# Autodesk Inventor assembly: 0005-00-02 X axis
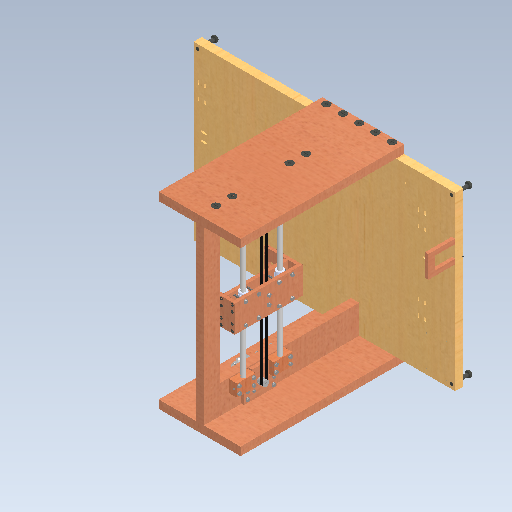
[picture p0: Inventor's stored thumbnail of the model, 512x512]
Saved by Autodesk Inventor 2020 (Build 240168000, 168)
## iProperties
Created: 2020-12-18
Part Number: 0005-00-02 X axis
Document SubType Name: Assembly
Designer: Iulian Bors
Mass: 798.511 g
Surface Area: 2520.75 cm^2
Volume: 569.854 cm^3
Density: 1.40126 g/cm^3
Author: Iulian Bors
Subject: 10-02
## Documents named in this file (22)
- Z:\I.A.B\Proiecte\0005 I.A.B 3d 2.0 Imprimanta aracet\10 Mecanic\0005-10-02 X axis.iam
- Z:\I.A.B\Proiecte\0005 I.A.B 3d 2.0 Imprimanta aracet\10 Mecanic\0005-10-011.ipt
- Z:\I.A.B\Proiecte\0005 I.A.B 3d 2.0 Imprimanta aracet\10 Mecanic\0005-10-012.ipt
- Z:\I.A.B\Proiecte\0005 I.A.B 3d 2.0 Imprimanta aracet\10 Mecanic\0005-10-1009 LM10uu.ipt
- Z:\I.A.B\Proiecte\0005 I.A.B 3d 2.0 Imprimanta aracet\10 Mecanic\Surub M4 saiba piulita.iam
- Z:\I.A.B\Proiecte\0005 I.A.B 3d 2.0 Imprimanta aracet\10 Mecanic\0005-10-1007 Bara rectificata.ipt
- Z:\I.A.B\Proiecte\0005 I.A.B 3d 2.0 Imprimanta aracet\10 Mecanic\0005-10-015 suport tija.ipt
- Z:\I.A.B\Proiecte\0005 I.A.B 3d 2.0 Imprimanta aracet\10 Mecanic\0005-10-1001 NEMA17 - Motor de passo.ipt
- Z:\I.A.B\Proiecte\0005 I.A.B 3d 2.0 Imprimanta aracet\10 Mecanic\0005-10-1010 GT2 Timing Pulley 20 Tooth.ipt
- Z:\I.A.B\Proiecte\0005 I.A.B 3d 2.0 Imprimanta aracet\10 Mecanic\0005-10-1011 16T W6 B3 Without T_Shrinkwrap_1.ipt
- Z:\I.A.B\Proiecte\0005 I.A.B 3d 2.0 Imprimanta aracet\10 Mecanic\0005-10-018 intinzator x.ipt
- Z:\I.A.B\Proiecte\0005 I.A.B 3d 2.0 Imprimanta aracet\10 Mecanic\0005-10-1015 curea x.ipt
- Z:\I.A.B\Proiecte\0005 I.A.B 3d 2.0 Imprimanta aracet\10 Mecanic\0005-10-023 Suport motor x.ipt
- Z:\I.A.B\Proiecte\0005 I.A.B 3d 2.0 Imprimanta aracet\10 Mecanic\Surub M4 saiba piulita 50mm.iam
- Z:\I.A.B\Proiecte\0005 I.A.B 3d 2.0 Imprimanta aracet\10 Mecanic\Surub M4 saiba piulita 60mm.iam
- Z:\I.A.B\Proiecte\0005 I.A.B 3d 2.0 Imprimanta aracet\10 Mecanic\0005-10-1032.ipt
- Z:\I.A.B\Proiecte\0005 I.A.B 3d 2.0 Imprimanta aracet\10 Mecanic\0005-10-1020 ISO 7089 - 3 - 140 HV(1).ipt
- Z:\I.A.B\Proiecte\0005 I.A.B 3d 2.0 Imprimanta aracet\10 Mecanic\0005-10-1033 DIN 914 - M5 x 10.ipt
- Z:\I.A.B\Proiecte\0005 I.A.B 3d 2.0 Imprimanta aracet\10 Mecanic\0005-10-027 suport nema Z.ipt
- Z:\I.A.B\Proiecte\0005 I.A.B 3d 2.0 Imprimanta aracet\10 Mecanic\0005-10-01 Cadru_Shrinkwrap_1.ipt
- Z:\I.A.B\Proiecte\0005 I.A.B 3d 2.0 Imprimanta aracet\10 Mecanic\0005-10-1045ISO 7050 - ST 3.5 x 22 - C - Z.ipt
- Z:\I.A.B\Proiecte\0005 I.A.B 3d 2.0 Imprimanta aracet\10 Mecanic\0005-10-1048 DIN 933 - M5  x 25.ipt
## Components (82 placed, 21 different names)
1. 0005-10-011.ipt:1 — Flush:69, Flush:70, Mate:151, Insert:33, Insert:34
2. 0005-10-027 suport nema Z.ipt:2 — Mate:142, Flush:71, Flush:72, Insert:35, Insert:36
3. 0005-10-012.ipt:3 — Flush:22, Flush:25, Flush:26, Mate:40, Mate:56, Mate:57, Mate:71, Mate:72, Flush:44, Mate:142, Mate:151
4. 0005-10-1009 LM10uu.ipt:4 — Flush:22, Mate:49, Mate:56, Mate:57
5. 0005-10-012.ipt:5 — Flush:25, Flush:34, Flush:26, Mate:40, Insert:18, Insert:19, Flush:69, Flush:70, Flush:71, Flush:72, Insert:21, Insert:22, Insert:24, Insert:25, Insert:27, Insert:28, Insert:30, Insert:40
6. 0005-10-1009 LM10uu.ipt:6 — Mate:49, Flush:34, Flush:45, Mate:172
7. 0005-10-1009 LM10uu.ipt:7 — Mate:71, Mate:72, Flush:44, Mate:73
8. 0005-10-1009 LM10uu.ipt:8 — Flush:45, Mate:73, Mate:164
9. Surub M4 saiba piulita.iam:9 [sub-assembly] — Insert:18
10. Surub M4 saiba piulita.iam:10 [sub-assembly] — Insert:19
11. Surub M4 saiba piulita.iam:11 [sub-assembly] — Insert:21
12. Surub M4 saiba piulita.iam:12 [sub-assembly] — Insert:22
13. Surub M4 saiba piulita.iam:13 [sub-assembly] — Insert:24
14. Surub M4 saiba piulita.iam:14 [sub-assembly] — Insert:27
15. Surub M4 saiba piulita.iam:15 [sub-assembly] — Insert:25
16. Surub M4 saiba piulita.iam:16 [sub-assembly] — Insert:28
17. Surub M4 saiba piulita.iam:17 [sub-assembly] — Insert:30
18. 0005-10-1007 Bara rectificata.ipt:18 — Mate:172, Mate:173, Flush:75, Mate:176, Flush:77
19. 0005-10-015 suport tija.ipt:19 — Mate:165, Mate:166, Mate:167, Mate:171, Flush:74, Flush:76, Insert:43, Insert:51
20. 0005-10-1001 NEMA17 - Motor de passo.ipt:20 — Insert:38, Angle:1
21. 0005-10-1010 GT2 Timing Pulley 20 Tooth.ipt:21
22. 0005-10-1011 16T W6 B3 Without T_Shrinkwrap_1.ipt:22 — Insert:39
23. 0005-10-018 intinzator x.ipt:23 — Mate:168, Mate:169, Mate:170, Insert:39, Insert:46, Insert:47, Insert:48
24. 0005-10-1015 curea x.ipt:24 — Angle:2
25. 0005-10-023 Suport motor x.ipt:25 — Insert:37, Mate:175, Insert:38, Insert:45, Insert:50
26. 0005-10-1007 Bara rectificata.ipt:42 — Mate:164, Mate:171, Flush:74, Mate:177, Flush:78
27. 0005-10-01 Cadru_Shrinkwrap_1.ipt:43 — Mate:165, Mate:166, Mate:167, Mate:170, Mate:174, Insert:37, Mate:175, Mate:178, Mate:179, Angle:2, Angle:3
28. 0005-10-015 suport tija.ipt:44 — Mate:173, Flush:75, Mate:174, Flush:76, Insert:44, Insert:52
29. Surub M4 saiba piulita.iam:45 [sub-assembly] — Insert:40
30. 0005-10-015 suport tija.ipt:46 — Mate:176, Flush:77, Mate:179, Insert:41, Insert:54
31. 0005-10-015 suport tija.ipt:47 — Mate:177, Flush:78, Mate:178, Insert:42, Insert:53
32. 0005-10-1048 DIN 933 - M5  x 25.ipt:68 — Insert:46
33. Surub M4 saiba piulita 60mm.iam:69 [sub-assembly] — Insert:48, Mate:168
34. Surub M4 saiba piulita 60mm.iam:70 [sub-assembly] — Insert:47, Mate:169
35. 0005-10-1033 DIN 914 - M5 x 10.ipt:79 — Insert:51
36. 0005-10-1033 DIN 914 - M5 x 10.ipt:80 — Insert:52
37. 0005-10-1033 DIN 914 - M5 x 10.ipt:81 — Insert:54
38. 0005-10-1033 DIN 914 - M5 x 10.ipt:82 — Insert:53
39. 0005-10-1045ISO 7050 - ST 3.5 x 22 - C - Z.ipt:26 — Insert:34
40. 0005-10-1045ISO 7050 - ST 3.5 x 22 - C - Z.ipt:27
41. 0005-10-1045ISO 7050 - ST 3.5 x 22 - C - Z.ipt:28
42. 0005-10-1045ISO 7050 - ST 3.5 x 22 - C - Z.ipt:29
43. 0005-10-1045ISO 7050 - ST 3.5 x 22 - C - Z.ipt:30 — Insert:33
44. 0005-10-1045ISO 7050 - ST 3.5 x 22 - C - Z.ipt:31
45. 0005-10-1045ISO 7050 - ST 3.5 x 22 - C - Z.ipt:32
46. 0005-10-1045ISO 7050 - ST 3.5 x 22 - C - Z.ipt:33
47. 0005-10-1045ISO 7050 - ST 3.5 x 22 - C - Z.ipt:34 — Insert:36
48. 0005-10-1045ISO 7050 - ST 3.5 x 22 - C - Z.ipt:35
49. 0005-10-1045ISO 7050 - ST 3.5 x 22 - C - Z.ipt:36
50. 0005-10-1045ISO 7050 - ST 3.5 x 22 - C - Z.ipt:37
51. 0005-10-1045ISO 7050 - ST 3.5 x 22 - C - Z.ipt:38 — Insert:35
52. 0005-10-1045ISO 7050 - ST 3.5 x 22 - C - Z.ipt:39
53. 0005-10-1045ISO 7050 - ST 3.5 x 22 - C - Z.ipt:40
54. 0005-10-1045ISO 7050 - ST 3.5 x 22 - C - Z.ipt:41
55. Surub M4 saiba piulita 50mm.iam:48 [sub-assembly] — Insert:41
56. Surub M4 saiba piulita 50mm.iam:49 [sub-assembly]
57. Surub M4 saiba piulita 50mm.iam:50 [sub-assembly]
58. Surub M4 saiba piulita 50mm.iam:51 [sub-assembly]
59. Surub M4 saiba piulita 50mm.iam:52 [sub-assembly] — Insert:42
60. Surub M4 saiba piulita 50mm.iam:53 [sub-assembly]
61. Surub M4 saiba piulita 50mm.iam:54 [sub-assembly]
62. Surub M4 saiba piulita 50mm.iam:55 [sub-assembly]
63. Surub M4 saiba piulita 50mm.iam:56 [sub-assembly] — Insert:43
64. Surub M4 saiba piulita 50mm.iam:57 [sub-assembly]
65. Surub M4 saiba piulita 50mm.iam:58 [sub-assembly]
66. Surub M4 saiba piulita 50mm.iam:59 [sub-assembly]
67. Surub M4 saiba piulita 50mm.iam:60 [sub-assembly] — Insert:44
68. Surub M4 saiba piulita 50mm.iam:61 [sub-assembly]
69. Surub M4 saiba piulita 50mm.iam:62 [sub-assembly]
70. Surub M4 saiba piulita 50mm.iam:63 [sub-assembly]
71. Surub M4 saiba piulita.iam:64 [sub-assembly] — Insert:45
72. Surub M4 saiba piulita.iam:65 [sub-assembly]
73. Surub M4 saiba piulita.iam:66 [sub-assembly] — Angle:3
74. Surub M4 saiba piulita.iam:67 [sub-assembly]
75. 0005-10-1032.ipt:71 — Insert:49
76. 0005-10-1020 ISO 7089 - 3 - 140 HV(1).ipt:72 — Insert:49, Insert:50
77. 0005-10-1032.ipt:73
78. 0005-10-1020 ISO 7089 - 3 - 140 HV(1).ipt:74
79. 0005-10-1032.ipt:75
80. 0005-10-1020 ISO 7089 - 3 - 140 HV(1).ipt:76
81. 0005-10-1032.ipt:77
82. 0005-10-1020 ISO 7089 - 3 - 140 HV(1).ipt:78
## Component patterns: (4 elements, first: 0005-10-1045ISO 7050 - ST 3.5 x 22 - C - Z.ipt:26), (4 elements, first: 0005-10-1045ISO 7050 - ST 3.5 x 22 - C - Z.ipt:30), (4 elements, first: 0005-10-1045ISO 7050 - ST 3.5 x 22 - C - Z.ipt:34), (4 elements, first: 0005-10-1045ISO 7050 - ST 3.5 x 22 - C - Z.ipt:38), (4 elements, first: Surub M4 saiba piulita 50mm.iam:48), (4 elements, first: Surub M4 saiba piulita 50mm.iam:52), (4 elements, first: Surub M4 saiba piulita 50mm.iam:56), (4 elements, first: Surub M4 saiba piulita 50mm.iam:60), (4 elements, first: Surub M4 saiba piulita.iam:64), (4 elements, first: 0005-10-1032.ipt:71 + 0005-10-1020 ISO 7089 - 3 - 140 HV(1).ipt:72)
## Relationships (79: Insert 31, Mate 29, Flush 16, Angle 3)
- Flush:22: 0005-10-012.ipt:3 ↔ 0005-10-1009 LM10uu.ipt:4
- Flush:25: 0005-10-012.ipt:3 ↔ 0005-10-012.ipt:5
- Flush:34: 0005-10-012.ipt:5 ↔ 0005-10-1009 LM10uu.ipt:6
- Flush:26: 0005-10-012.ipt:3 ↔ 0005-10-012.ipt:5
- Mate:40 (19 mm): 0005-10-012.ipt:3 ↔ 0005-10-012.ipt:5
- Mate:49: 0005-10-1009 LM10uu.ipt:4 ↔ 0005-10-1009 LM10uu.ipt:6
- Mate:56 (9.5 mm): 0005-10-012.ipt:3 ↔ 0005-10-1009 LM10uu.ipt:4
- Mate:57 (-30 mm): 0005-10-012.ipt:3 ↔ 0005-10-1009 LM10uu.ipt:4
- Mate:71: 0005-10-012.ipt:3 ↔ 0005-10-1009 LM10uu.ipt:7
- Mate:72 (9.5 mm): 0005-10-012.ipt:3 ↔ 0005-10-1009 LM10uu.ipt:7
- Flush:44 (30 mm): 0005-10-012.ipt:3 ↔ 0005-10-1009 LM10uu.ipt:7
- Flush:45: 0005-10-1009 LM10uu.ipt:6 ↔ 0005-10-1009 LM10uu.ipt:8
- Mate:73: 0005-10-1009 LM10uu.ipt:7 ↔ 0005-10-1009 LM10uu.ipt:8
- Insert:18: 0005-10-012.ipt:5 ↔ Surub M4 saiba piulita.iam:9
- Insert:19: 0005-10-012.ipt:5 ↔ Surub M4 saiba piulita.iam:10
- Flush:69: 0005-10-011.ipt:1 ↔ 0005-10-012.ipt:5
- Flush:70: 0005-10-011.ipt:1 ↔ 0005-10-012.ipt:5
- Mate:142: 0005-10-027 suport nema Z.ipt:2 ↔ 0005-10-012.ipt:3
- Flush:71: 0005-10-027 suport nema Z.ipt:2 ↔ 0005-10-012.ipt:5
- Flush:72: 0005-10-027 suport nema Z.ipt:2 ↔ 0005-10-012.ipt:5
- Mate:151: 0005-10-011.ipt:1 ↔ 0005-10-012.ipt:3
- Insert:21: 0005-10-012.ipt:5 ↔ Surub M4 saiba piulita.iam:11
- Insert:22: 0005-10-012.ipt:5 ↔ Surub M4 saiba piulita.iam:12
- Insert:24: 0005-10-012.ipt:5 ↔ Surub M4 saiba piulita.iam:13
- Insert:25: 0005-10-012.ipt:5 ↔ Surub M4 saiba piulita.iam:15
- Insert:27: 0005-10-012.ipt:5 ↔ Surub M4 saiba piulita.iam:14
- Insert:28: 0005-10-012.ipt:5 ↔ Surub M4 saiba piulita.iam:16
- Insert:30: 0005-10-012.ipt:5 ↔ Surub M4 saiba piulita.iam:17
- [Flush]: 0005-10-1010 GT2 Timing Pulley 20 Tooth.ipt:21 ↔ 0005-10-1011 16T W6 B3 Without T_Shrinkwrap_1.ipt:22
- [Mate]: 0005-10-1010 GT2 Timing Pulley 20 Tooth.ipt:21 ↔ 0005-10-1011 16T W6 B3 Without T_Shrinkwrap_1.ipt:22
- [Mate]: 0005-10-1010 GT2 Timing Pulley 20 Tooth.ipt:21 ↔ 0005-10-1015 curea x.ipt:24
- [Mate]: 0005-10-1010 GT2 Timing Pulley 20 Tooth.ipt:21 ↔ 0005-10-1015 curea x.ipt:24
- [Mate]: 0005-10-1001 NEMA17 - Motor de passo.ipt:20 ↔ 0005-10-1010 GT2 Timing Pulley 20 Tooth.ipt:21
- Insert:33: 0005-10-011.ipt:1 ↔ 0005-10-1045ISO 7050 - ST 3.5 x 22 - C - Z.ipt:30
- Insert:34: 0005-10-011.ipt:1 ↔ 0005-10-1045ISO 7050 - ST 3.5 x 22 - C - Z.ipt:26
- Insert:35: 0005-10-027 suport nema Z.ipt:2 ↔ 0005-10-1045ISO 7050 - ST 3.5 x 22 - C - Z.ipt:38
- Insert:36: 0005-10-027 suport nema Z.ipt:2 ↔ 0005-10-1045ISO 7050 - ST 3.5 x 22 - C - Z.ipt:34
- Mate:164: 0005-10-1009 LM10uu.ipt:8 ↔ 0005-10-1007 Bara rectificata.ipt:42
- Mate:165: 0005-10-015 suport tija.ipt:19 ↔ 0005-10-01 Cadru_Shrinkwrap_1.ipt:43
- Mate:166: 0005-10-015 suport tija.ipt:19 ↔ 0005-10-01 Cadru_Shrinkwrap_1.ipt:43
- Mate:167: 0005-10-015 suport tija.ipt:19 ↔ 0005-10-01 Cadru_Shrinkwrap_1.ipt:43
- Mate:168: 0005-10-018 intinzator x.ipt:23 ↔ Surub M4 saiba piulita 60mm.iam:69
- Mate:169: 0005-10-018 intinzator x.ipt:23 ↔ Surub M4 saiba piulita 60mm.iam:70
- Mate:170: 0005-10-018 intinzator x.ipt:23 ↔ 0005-10-01 Cadru_Shrinkwrap_1.ipt:43
- Mate:171: 0005-10-015 suport tija.ipt:19 ↔ 0005-10-1007 Bara rectificata.ipt:42
- Flush:74: 0005-10-015 suport tija.ipt:19 ↔ 0005-10-1007 Bara rectificata.ipt:42
- Mate:172: 0005-10-1009 LM10uu.ipt:6 ↔ 0005-10-1007 Bara rectificata.ipt:18
- Mate:173: 0005-10-1007 Bara rectificata.ipt:18 ↔ 0005-10-015 suport tija.ipt:44
- Flush:75: 0005-10-1007 Bara rectificata.ipt:18 ↔ 0005-10-015 suport tija.ipt:44
- Mate:174: 0005-10-01 Cadru_Shrinkwrap_1.ipt:43 ↔ 0005-10-015 suport tija.ipt:44
- Flush:76: 0005-10-015 suport tija.ipt:19 ↔ 0005-10-015 suport tija.ipt:44
- Insert:37: 0005-10-023 Suport motor x.ipt:25 ↔ 0005-10-01 Cadru_Shrinkwrap_1.ipt:43
- Mate:175: 0005-10-023 Suport motor x.ipt:25 ↔ 0005-10-01 Cadru_Shrinkwrap_1.ipt:43
- Insert:38: 0005-10-1001 NEMA17 - Motor de passo.ipt:20 ↔ 0005-10-023 Suport motor x.ipt:25
- Angle:1 (0 deg): 0005-10-1001 NEMA17 - Motor de passo.ipt:20
- Insert:39 (1 mm): 0005-10-1011 16T W6 B3 Without T_Shrinkwrap_1.ipt:22 ↔ 0005-10-018 intinzator x.ipt:23
- Insert:40: 0005-10-012.ipt:5 ↔ Surub M4 saiba piulita.iam:45
- Mate:176: 0005-10-1007 Bara rectificata.ipt:18 ↔ 0005-10-015 suport tija.ipt:46
- Flush:77: 0005-10-1007 Bara rectificata.ipt:18 ↔ 0005-10-015 suport tija.ipt:46
- Mate:177: 0005-10-1007 Bara rectificata.ipt:42 ↔ 0005-10-015 suport tija.ipt:47
- Flush:78: 0005-10-1007 Bara rectificata.ipt:42 ↔ 0005-10-015 suport tija.ipt:47
- Mate:178: 0005-10-01 Cadru_Shrinkwrap_1.ipt:43 ↔ 0005-10-015 suport tija.ipt:47
- Mate:179: 0005-10-01 Cadru_Shrinkwrap_1.ipt:43 ↔ 0005-10-015 suport tija.ipt:46
- Insert:41: 0005-10-015 suport tija.ipt:46 ↔ Surub M4 saiba piulita 50mm.iam:48
- Insert:42: 0005-10-015 suport tija.ipt:47 ↔ Surub M4 saiba piulita 50mm.iam:52
- Insert:43: 0005-10-015 suport tija.ipt:19 ↔ Surub M4 saiba piulita 50mm.iam:56
- Insert:44: 0005-10-015 suport tija.ipt:44 ↔ Surub M4 saiba piulita 50mm.iam:60
- Angle:2 (0 deg): 0005-10-1015 curea x.ipt:24 ↔ 0005-10-01 Cadru_Shrinkwrap_1.ipt:43
- Insert:45: 0005-10-023 Suport motor x.ipt:25 ↔ Surub M4 saiba piulita.iam:64
- Insert:46: 0005-10-018 intinzator x.ipt:23 ↔ 0005-10-1048 DIN 933 - M5  x 25.ipt:68
- Insert:47: 0005-10-018 intinzator x.ipt:23 ↔ Surub M4 saiba piulita 60mm.iam:70
- Insert:48: 0005-10-018 intinzator x.ipt:23 ↔ Surub M4 saiba piulita 60mm.iam:69
- Insert:49: 0005-10-1032.ipt:71 ↔ 0005-10-1020 ISO 7089 - 3 - 140 HV(1).ipt:72
- Insert:50: 0005-10-023 Suport motor x.ipt:25 ↔ 0005-10-1020 ISO 7089 - 3 - 140 HV(1).ipt:72
- Angle:3 (0 deg): 0005-10-01 Cadru_Shrinkwrap_1.ipt:43 ↔ Surub M4 saiba piulita.iam:66
- Insert:51: 0005-10-015 suport tija.ipt:19 ↔ 0005-10-1033 DIN 914 - M5 x 10.ipt:79
- Insert:52: 0005-10-015 suport tija.ipt:44 ↔ 0005-10-1033 DIN 914 - M5 x 10.ipt:80
- Insert:53: 0005-10-015 suport tija.ipt:47 ↔ 0005-10-1033 DIN 914 - M5 x 10.ipt:82
- Insert:54: 0005-10-015 suport tija.ipt:46 ↔ 0005-10-1033 DIN 914 - M5 x 10.ipt:81
